# Autodesk Inventor assembly: rev6
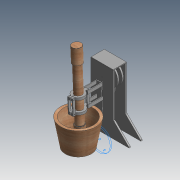
[picture p0: Inventor's stored thumbnail of the model, 180x180]
Saved by Autodesk Inventor 2015 (Build 190159000, 159)
## iProperties
Created: 2014-08-31
Part Number: rev6
Document SubType Name: Assembly
Designer: shohei
Author: shohei
## Documents named in this file (25)
- C:\Users\shohei\Documents\Inventor\FufuPounderGeared\rev6.iam
- C:\Users\shohei\Documents\Inventor\FufuPounderGeared\mortar2.ipt
- C:\Users\shohei\Documents\Inventor\FufuPounderGeared\sideplate.ipt
- C:\Users\shohei\Documents\Inventor\FufuPounderGeared\mainpulley.ipt
- C:\Users\shohei\Documents\Inventor\FufuPounderGeared\drivepulley.ipt
- C:\Users\shohei\Documents\Inventor\FufuPounderGeared\shaft5.ipt
- C:\Users\shohei\Documents\Inventor\FufuPounderGeared\drivelever.ipt
- C:\Users\shohei\Documents\Inventor\FufuPounderGeared\shaft7.ipt
- C:\Users\shohei\Documents\Inventor\FufuPounderGeared\globals.ipt
- C:\Users\shohei\Documents\Inventor\FufuPounderGeared\shaft8.ipt
- C:\Users\shohei\Documents\Inventor\FufuPounderGeared\shaft9.ipt
- C:\Users\shohei\Documents\Inventor\FufuPounderGeared\mallet_new.ipt
- C:\Users\shohei\Documents\Inventor\FufuPounderGeared\mallet_holder.ipt
- C:\Users\shohei\Documents\Inventor\FufuPounderGeared\mallet_sideplate.ipt
- C:\Users\shohei\Documents\Inventor\FufuPounderGeared\holderBlock.ipt
- C:\Users\shohei\Documents\Inventor\FufuPounderGeared\sideplate_top.ipt
- C:\Users\shohei\Documents\Inventor\FufuPounderGeared\shaft10.ipt
- C:\Users\shohei\Documents\Inventor\FufuPounderGeared\holderBlock2.ipt
- C:\Users\shohei\Documents\Inventor\FufuPounderGeared\gripsupport.ipt
- C:\Users\shohei\Documents\Inventor\FufuPounder\rev6\AIP\FEA\b5u4ebwdc.fins
- C:\Users\shohei\Documents\Inventor\FufuPounder\rev6\AIP\FEA\b5u4ebwdc.fsat
- C:\Users\shohei\Documents\Inventor\FufuPounder\rev6\AIP\FEA\b5u4ebwdc.ftes
- C:\Users\shohei\Documents\Inventor\FufuPounder\rev6\AIP\FEA\b5u4ebwdc.fwiz
- C:\Users\shohei\Documents\Inventor\FufuPounder\rev6\AIP\FEA\b5u4ebwgw.fmsh
- C:\Users\shohei\Documents\Inventor\FufuPounder\rev6\AIP\FEA\b5u4ebwgx.fres
## Components (27 placed, 18 different names)
1. mortar2:1 — Mate:1
2. sideplate:1 — Mate:2, Flush:1, Slider:1, Mate:9, Flush:13, Flush:14, Rotational:17
3. sideplate:2 — Mate:3, Flush:1, Rotational:10, Flush:15, Slider:2
4. mainpulley:1 — Rotational:4, Angle:1, Rotational:15
5. drivepulley:1 — Rotational:16
6. shaft5:2 — Rotational:4, Rotational:8
7. drivelever:1 — Cylindrical:1, Rotational:8
8. shaft7:1 — Slider:1, Cylindrical:1, Rotational:14, Rotational:18
9. globals:1
10. mainpulley:2 — Rotational:9
11. shaft8:1 — Rotational:9, Rotational:10
12. shaft9:2 — Cylindrical:4, Cylindrical:5, Slider:2
13. mallet_new:1 — Rigid:1
14. mallet_holder:1 — Flush:3, Mate:5, Flush:4, Mate:6, Flush:5, Flush:6, Flush:9, Mate:7, Flush:10, Mate:8, Flush:11, Flush:12, Rigid:1
15. mallet_holder:2 — Flush:7, Mate:15
16. mallet_sideplate:1 — Flush:3, Mate:5, Flush:4, Flush:7, Flush:22, Flush:23, Mate:13, Flush:27, Mate:15
17. mallet_sideplate:2 — Flush:9, Mate:7, Flush:10
18. mallet_sideplate:3 — Mate:6, Flush:5, Flush:6, Flush:20, Flush:21, Mate:12, Mate:14, Flush:25, Flush:26
19. mallet_sideplate:4 — Mate:8, Flush:11, Flush:12
20. holderBlock:2 — Rotational:14, Cylindrical:4
21. sideplate_top:1 — Mate:9, Flush:13, Flush:14, Flush:15
22. shaft10:1 — Rotational:15, Rotational:16, Rotational:17
23. holderBlock2:1 — Rotational:18, Cylindrical:5, Mate:10, Mate:11, Flush:16, Flush:17, Flush:18, Flush:19, Flush:24
24. gripsupport:1 — Mate:11, Flush:16, Flush:19, Flush:22, Flush:23
25. gripsupport:2 — Mate:10, Flush:17, Flush:18, Flush:20, Flush:21, Mate:12
26. gripsupport:3 — Mate:13, Flush:24, Flush:27
27. gripsupport:4 — Mate:14, Flush:25, Flush:26
## Relationships (55: Flush 25, Mate 14, RevoluteJoint 9, CylindricalJoint 3, TranslationJoint 2, Angle 1, WeldJoint 1)
- Mate:1: mortar2:1
- Rotational:4 [RevoluteJoint]: mainpulley:1 ↔ shaft5:2
- Mate:2: sideplate:1
- Mate:3: sideplate:2
- Flush:1: sideplate:1 ↔ sideplate:2
- Slider:1 [TranslationJoint]: sideplate:1 ↔ shaft7:1
- Cylindrical:1: drivelever:1 ↔ shaft7:1
- Rotational:8 [RevoluteJoint] (-30 mm): shaft5:2 ↔ drivelever:1
- Angle:1 (270 deg): mainpulley:1
- Rotational:9 [RevoluteJoint]: mainpulley:2 ↔ shaft8:1
- Rotational:10 [RevoluteJoint]: sideplate:2 ↔ shaft8:1
- Flush:3: mallet_holder:1 ↔ mallet_sideplate:1
- Mate:5: mallet_holder:1 ↔ mallet_sideplate:1
- Flush:4: mallet_holder:1 ↔ mallet_sideplate:1
- Mate:6: mallet_holder:1 ↔ mallet_sideplate:3
- Flush:5: mallet_holder:1 ↔ mallet_sideplate:3
- Flush:6: mallet_holder:1 ↔ mallet_sideplate:3
- Flush:7: mallet_holder:2 ↔ mallet_sideplate:1
- Flush:9: mallet_holder:1 ↔ mallet_sideplate:2
- Mate:7: mallet_holder:1 ↔ mallet_sideplate:2
- Flush:10: mallet_holder:1 ↔ mallet_sideplate:2
- Mate:8: mallet_holder:1 ↔ mallet_sideplate:4
- Flush:11: mallet_holder:1 ↔ mallet_sideplate:4
- Flush:12: mallet_holder:1 ↔ mallet_sideplate:4
- Rotational:14 [RevoluteJoint] (-30 mm): shaft7:1 ↔ holderBlock:2
- Cylindrical:4: shaft9:2 ↔ holderBlock:2
- Mate:9: sideplate:1 ↔ sideplate_top:1
- Flush:13: sideplate:1 ↔ sideplate_top:1
- Flush:14: sideplate:1 ↔ sideplate_top:1
- Rotational:15 [RevoluteJoint]: mainpulley:1 ↔ shaft10:1
- Rotational:16 [RevoluteJoint]: drivepulley:1 ↔ shaft10:1
- Flush:15: sideplate:2 ↔ sideplate_top:1
- Rotational:17 [RevoluteJoint] (-80 mm): sideplate:1 ↔ shaft10:1
- Rotational:18 [RevoluteJoint]: shaft7:1 ↔ holderBlock2:1
- Cylindrical:5: shaft9:2 ↔ holderBlock2:1
- Mate:10: holderBlock2:1 ↔ gripsupport:2
- Mate:11: holderBlock2:1 ↔ gripsupport:1
- Flush:16: holderBlock2:1 ↔ gripsupport:1
- Flush:17: holderBlock2:1 ↔ gripsupport:2
- Flush:18: holderBlock2:1 ↔ gripsupport:2
- Flush:19: holderBlock2:1 ↔ gripsupport:1
- Flush:20: mallet_sideplate:3 ↔ gripsupport:2
- Flush:21: mallet_sideplate:3 ↔ gripsupport:2
- Flush:22: mallet_sideplate:1 ↔ gripsupport:1
- Flush:23: mallet_sideplate:1 ↔ gripsupport:1
- Mate:12: mallet_sideplate:3 ↔ gripsupport:2
- Mate:13: mallet_sideplate:1 ↔ gripsupport:3
- Flush:24: holderBlock2:1 ↔ gripsupport:3
- Mate:14: mallet_sideplate:3 ↔ gripsupport:4
- Flush:25: mallet_sideplate:3 ↔ gripsupport:4
- Flush:26: mallet_sideplate:3 ↔ gripsupport:4
- Flush:27: mallet_sideplate:1 ↔ gripsupport:3
- Mate:15: mallet_holder:2 ↔ mallet_sideplate:1
- Rigid:1 [WeldJoint]: mallet_new:1 ↔ mallet_holder:1
- Slider:2 [TranslationJoint]: sideplate:2 ↔ shaft9:2
## Named parameters: sa_0 = 0, sa_1 = 3.2e-12, sa_2 = 10000
note: some values were not read from the file. Shown as the stored number, unit unknown: "sa_0", "sa_1", "sa_2".
